# Autodesk Inventor assembly: Motor_assembly
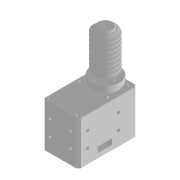
[picture p0: Inventor's stored thumbnail of the model, 180x180]
Saved by Autodesk Inventor 2022 (Build 260153000, 153)
## iProperties
Created: 2022-07-07
Part Number: Motor_assembly
Document SubType Name: Assembly
Designer: dell
Author: dell
## Documents named in this file (5)
- D:\xxxx\Uni\Part IV\MECHENG_700\Part_IV_project_CAD\Bird_skeleton_prototypes\Wing_drone_V1\Bird_wing_V1\Motor_assembly.iam
- D:\xxxx\Uni\Part IV\MECHENG_700\Part_IV_project_CAD\Bird_skeleton_prototypes\Wing_drone_V1\Bird_wing_V1\Worm_1.0_module\57545K617_Shaft-Mounted Worm.ipt
- D:\xxxx\Uni\Part IV\MECHENG_700\Part_IV_project_CAD\Bird_skeleton_prototypes\Wing_drone_V1\XM430.iam
- D:\xxxx\Uni\Part IV\MECHENG_700\Part_IV_project_CAD\Bird_skeleton_prototypes\Wing_drone_V1\Bird_wing_V1\XM430_motor_adaptor.ipt
- D:\xxxx\Uni\Part IV\MECHENG_700\Part_IV_project_CAD\Bird_skeleton_prototypes\Wing_drone_V1\Bird_wing_V1\XM430_motor_adaptor_cap.ipt
## Components (4 placed, 4 different names)
1. 57545K617_Shaft-Mounted Worm:1 — Mate:4, Mate:5, Mate:6, Mate:7
2. XM430:1 [sub-assembly] — Mate:1, Mate:2, Mate:3
3. XM430_motor_adaptor:1 — Mate:1, Mate:2, Mate:3, Mate:4, Mate:5, Mate:6, Mate:8
4. XM430_motor_adaptor_cap:1 — Mate:7, Mate:8
## Relationships (8: Mate 8)
- Mate:1: XM430:1 ↔ XM430_motor_adaptor:1
- Mate:2: XM430:1 ↔ XM430_motor_adaptor:1
- Mate:3: XM430:1 ↔ XM430_motor_adaptor:1
- Mate:4 (0.1 mm): 57545K617_Shaft-Mounted Worm:1 ↔ XM430_motor_adaptor:1
- Mate:5 (0.1 mm): 57545K617_Shaft-Mounted Worm:1 ↔ XM430_motor_adaptor:1
- Mate:6 (1.5 mm): 57545K617_Shaft-Mounted Worm:1 ↔ XM430_motor_adaptor:1
- Mate:7: 57545K617_Shaft-Mounted Worm:1 ↔ XM430_motor_adaptor_cap:1
- Mate:8: XM430_motor_adaptor:1 ↔ XM430_motor_adaptor_cap:1
